# Autodesk Inventor assembly: Ensamble2
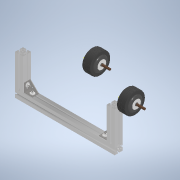
[picture p0: Inventor's stored thumbnail of the model, 180x180]
Saved by Autodesk Inventor 2021 (Build 250183000, 183)
## iProperties
Created: 2020-11-09
Part Number: Ensamble2
Document SubType Name: Assembly
Designer: juanm
Author: juanm
## Documents named in this file (7)
- C:\Users\juanm\OneDrive\Documentos\Inventor\NombreProyecto\Ensamble2.iam
- C:\Users\juanm\OneDrive\Documentos\Inventor\NombreProyecto\Horizontal.ipt
- C:\Users\juanm\OneDrive\Documentos\Inventor\NombreProyecto\Vertical.ipt
- C:\Users\juanm\OneDrive\Documentos\Inventor\NombreProyecto\Tornillo.ipt
- C:\Users\juanm\OneDrive\Documentos\Inventor\NombreProyecto\Sujetador2.ipt
- C:\Users\juanm\OneDrive\Documentos\Inventor\NombreProyecto\Tuerca para tornillo.ipt
- C:\Users\juanm\OneDrive\Documentos\Inventor\NombreProyecto\Llanta.ipt
## Components (15 placed, 6 different names)
1. Horizontal:1 — Nivelación:1, Nivelación:2, Coincidencia:1, Coincidencia:5, Coincidencia:7, Nivelación:3, Coincidencia:8, Coincidencia:9, Coincidencia:11, Nivelación:4, Nivelación:5, Coincidencia:15, Coincidencia:16, Coincidencia:18, Coincidencia:20, Nivelación:6
2. Vertical:2 — Nivelación:1, Nivelación:2, Coincidencia:1, Coincidencia:3, Coincidencia:4, Coincidencia:6, Coincidencia:10
3. Tornillo:1 — Coincidencia:8, Coincidencia:9, Coincidencia:10, De rotación:2
4. Tornillo:2 — Coincidencia:3, Coincidencia:4, Coincidencia:5, De rotación:1
5. Sujetador2:1 — Coincidencia:6, Coincidencia:7, Nivelación:3
6. Tuerca para tornillo:1 — De rotación:2
7. Tuerca para tornillo:2 — De rotación:1
8. Vertical:3 — Coincidencia:11, Nivelación:4, Nivelación:5, Coincidencia:13, Coincidencia:14, Coincidencia:19, Coincidencia:21
9. Sujetador2:2 — Coincidencia:20, Coincidencia:21, Nivelación:6
10. Tornillo:3 — Coincidencia:13, Coincidencia:14, Coincidencia:15, De rotación:4
11. Tornillo:4 — Coincidencia:16, Coincidencia:18, Coincidencia:19, De rotación:3
12. Tuerca para tornillo:3 — De rotación:3
13. Tuerca para tornillo:4 — De rotación:4
14. Llanta:1
15. Llanta:2
## Relationships (28: Mate 18, Flush 6, RevoluteJoint 4)
- Nivelación:1 [Flush]: Horizontal:1 ↔ Vertical:2
- Nivelación:2 [Flush]: Horizontal:1 ↔ Vertical:2
- Coincidencia:1 [Mate]: Horizontal:1 ↔ Vertical:2
- Coincidencia:3 [Mate]: Vertical:2 ↔ Tornillo:2
- Coincidencia:4 [Mate] (2.3 mm): Vertical:2 ↔ Tornillo:2
- Coincidencia:5 [Mate] (24 mm): Horizontal:1 ↔ Tornillo:2
- Coincidencia:6 [Mate]: Vertical:2 ↔ Sujetador2:1
- Coincidencia:7 [Mate]: Horizontal:1 ↔ Sujetador2:1
- Nivelación:3 [Flush] (5 mm): Horizontal:1 ↔ Sujetador2:1
- Coincidencia:8 [Mate]: Horizontal:1 ↔ Tornillo:1
- Coincidencia:9 [Mate] (2.3 mm): Horizontal:1 ↔ Tornillo:1
- Coincidencia:10 [Mate] (24 mm): Vertical:2 ↔ Tornillo:1
- De rotación:1 [RevoluteJoint] (7 mm): Tornillo:2 ↔ Tuerca para tornillo:2
- De rotación:2 [RevoluteJoint] (-7 mm): Tornillo:1 ↔ Tuerca para tornillo:1
- Coincidencia:11 [Mate]: Horizontal:1 ↔ Vertical:3
- Nivelación:4 [Flush]: Horizontal:1 ↔ Vertical:3
- Nivelación:5 [Flush]: Horizontal:1 ↔ Vertical:3
- Coincidencia:13 [Mate]: Vertical:3 ↔ Tornillo:3
- Coincidencia:14 [Mate] (2.3 mm): Vertical:3 ↔ Tornillo:3
- Coincidencia:15 [Mate] (24 mm): Horizontal:1 ↔ Tornillo:3
- Coincidencia:16 [Mate]: Horizontal:1 ↔ Tornillo:4
- Coincidencia:18 [Mate] (2.3 mm): Horizontal:1 ↔ Tornillo:4
- Coincidencia:19 [Mate] (24 mm): Vertical:3 ↔ Tornillo:4
- Coincidencia:20 [Mate]: Horizontal:1 ↔ Sujetador2:2
- Coincidencia:21 [Mate]: Vertical:3 ↔ Sujetador2:2
- Nivelación:6 [Flush] (5 mm): Horizontal:1 ↔ Sujetador2:2
- De rotación:3 [RevoluteJoint] (-15 mm): Tornillo:4 ↔ Tuerca para tornillo:3
- De rotación:4 [RevoluteJoint] (15 mm): Tornillo:3 ↔ Tuerca para tornillo:4
